# Autodesk Inventor assembly: Rulliera - Trasporto
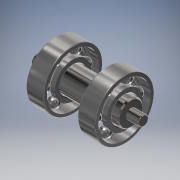
[picture p0: Inventor's stored thumbnail of the model, 180x180]
Saved by Autodesk Inventor 2018 (Build 220112000, 112)
## iProperties
Created: 2020-05-30
Part Number: Rulliera - Trasporto
Material: Generico
Document SubType Name: Assembly
Designer: Francesco
Author: Francesco
## Documents named in this file (3)
- C:\Users\Francesco\no-brim\Meccanica\Progetto Inventor no-brim\Assiemi\Rulliera - Trasporto.iam
- C:\Users\Francesco\no-brim\Meccanica\Progetto Inventor no-brim\Parti\Albero cuscinetto.ipt
- C:\Users\Francesco\no-brim\Meccanica\Progetto Inventor no-brim\Unificati\it-IT\SKF B - angular contact\SKF B7204 BE.ipt
## Components (3 placed, 2 different names)
1. Albero cuscinetto:1 — Coincidente:1, Allineato:1, Coincidente:2, Allineato:2
2. SKF B- Contatto angolare SKF B7204 BE:1 — Coincidente:1, Allineato:1
3. SKF B- Contatto angolare SKF B7204 BE:2 — Coincidente:2, Allineato:2
## Relationships (4: Mate 2, Flush 2)
- Coincidente:1 [Mate]: Albero cuscinetto:1 ↔ SKF B- Contatto angolare SKF B7204 BE:1
- Allineato:1 [Flush] (-5 mm): Albero cuscinetto:1 ↔ SKF B- Contatto angolare SKF B7204 BE:1
- Coincidente:2 [Mate]: Albero cuscinetto:1 ↔ SKF B- Contatto angolare SKF B7204 BE:2
- Allineato:2 [Flush] (5 mm): Albero cuscinetto:1 ↔ SKF B- Contatto angolare SKF B7204 BE:2
